# Autodesk Inventor assembly: Horizontal Grabber
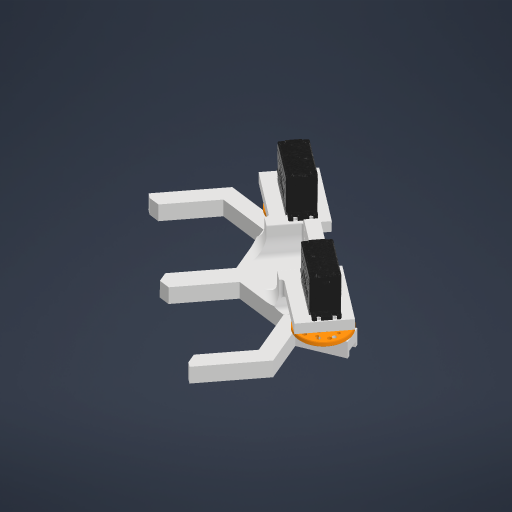
[picture p0: Inventor's stored thumbnail of the model, 512x512]
Saved by Autodesk Inventor 2024.2 (Build 282272000, 272)
## iProperties
Created: 2024-03-01
Part Number: Horizontal Grabber
Document SubType Name: Assembly
Designer: Jared
Author: Jared
## Documents named in this file (7)
- C:\Users\alniles07\Documents\Github\8400_2024_CAD\Horizontal Grabber.iam
- C:\Users\alniles07\Documents\Github\8400_2024_CAD\HorizontalGrabberMain.ipt
- C:\Users\alniles07\Documents\Github\8400_2024_CAD\HorizGrabberMoving.ipt
- C:\Users\alniles07\Documents\Github\8400_2024_CAD\Hex.ipt
- C:\Users\alniles07\Documents\Github\8400_2024_CAD\Servo Horn.ipt
- C:\Users\alniles07\Documents\Github\8400_2024_CAD\Smart Servo.ipt
- C:\Users\alniles07\Documents\Github\8400_2024_CAD\HorizGrabberMovingMirro.ipt
## Components (8 placed, 6 different names)
1. HorizontalGrabberMain:1 — Mate:1, Flush:1, Mate:2, Flush:2, Mate:3, Mate:20, Mate:23, Mate:26, Mate:29, Mate:32, Mate:35, Mate:37, Angle:1, Mate:38, Mate:42, Mate:43, Mate:45, Flush:4
2. HorizGrabberMoving:1 — Mate:1, Flush:1, Mate:3, Mate:5, Mate:8, Mate:11, Mate:14, Mate:17
3. Hex:1
4. Servo Horn:1 — Insert:1, Mate:4, Mate:7, Mate:10, Mate:13, Mate:16
5. Smart Servo:1 — Mate:2, Insert:1, Flush:2, Mate:19, Mate:22, Mate:25, Mate:28, Mate:31, Mate:34
6. Smart Servo:2 — Mate:38, Mate:41, Flush:3, Mate:42, Mate:43
7. Servo Horn:2 — Mate:41, Flush:3, Mate:44, Mate:46
8. HorizGrabberMovingMirro:1 — Mate:44, Mate:45, Flush:4, Mate:46
## Relationships (50: Mate 44, Flush 4, Insert 1, Angle 1)
- Mate:1: HorizontalGrabberMain:1 ↔ HorizGrabberMoving:1
- Flush:1: HorizontalGrabberMain:1 ↔ HorizGrabberMoving:1
- Mate:2: HorizontalGrabberMain:1 ↔ Smart Servo:1
- Insert:1: Servo Horn:1 ↔ Smart Servo:1
- Flush:2: HorizontalGrabberMain:1 ↔ Smart Servo:1
- Mate:3: HorizontalGrabberMain:1 ↔ HorizGrabberMoving:1
- Mate:4: Servo Horn:1
- Mate:5: HorizGrabberMoving:1
- Mate:6
- Mate:7: Servo Horn:1
- Mate:8: HorizGrabberMoving:1
- Mate:9
- Mate:10: Servo Horn:1
- Mate:11: HorizGrabberMoving:1
- Mate:12
- Mate:13: Servo Horn:1
- Mate:14: HorizGrabberMoving:1
- Mate:15
- Mate:16: Servo Horn:1
- Mate:17: HorizGrabberMoving:1
- Mate:18
- Mate:19: Smart Servo:1
- Mate:20: HorizontalGrabberMain:1
- Mate:21
- Mate:22: Smart Servo:1
- Mate:23: HorizontalGrabberMain:1
- Mate:24
- Mate:25: Smart Servo:1
- Mate:26: HorizontalGrabberMain:1
- Mate:27
- Mate:28: Smart Servo:1
- Mate:29: HorizontalGrabberMain:1
- Mate:30
- Mate:31: Smart Servo:1
- Mate:32: HorizontalGrabberMain:1
- Mate:33
- Mate:34: Smart Servo:1
- Mate:35: HorizontalGrabberMain:1
- Mate:36
- Mate:37: HorizontalGrabberMain:1
- Angle:1 (90 deg): HorizontalGrabberMain:1
- Mate:38: HorizontalGrabberMain:1 ↔ Smart Servo:2
- Mate:41: Smart Servo:2 ↔ Servo Horn:2
- Flush:3: Smart Servo:2 ↔ Servo Horn:2
- Mate:42: HorizontalGrabberMain:1 ↔ Smart Servo:2
- Mate:43: HorizontalGrabberMain:1 ↔ Smart Servo:2
- Mate:44: Servo Horn:2 ↔ HorizGrabberMovingMirro:1
- Mate:45: HorizontalGrabberMain:1 ↔ HorizGrabberMovingMirro:1
- Flush:4: HorizontalGrabberMain:1 ↔ HorizGrabberMovingMirro:1
- Mate:46: Servo Horn:2 ↔ HorizGrabberMovingMirro:1
